# Autodesk Inventor assembly: ElectricalBoxAssembly
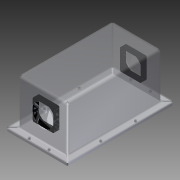
[picture p0: Inventor's stored thumbnail of the model, 180x180]
Saved by Autodesk Inventor 2015 (Build 190159000, 159)
## iProperties
Created: 2015-05-12
Part Number: ElectricalBoxAssembly
Document SubType Name: Assembly
Designer: carpenma
Author: carpenma
## Documents named in this file (4)
- C:\Users\carpe_000\Documents\GitHub\PFPRobot\Mechanical\Drivetrain WIth Cart\Electrical Board-Box\ElectricalBoxAssembly.iam
- C:\Users\carpe_000\Documents\GitHub\PFPRobot\Mechanical\Drivetrain WIth Cart\Electrical Board-Box\60mm Fan Footprint.ipt
- C:\Users\carpe_000\Documents\GitHub\PFPRobot\Mechanical\Drivetrain WIth Cart\Electrical Board-Box\Cover.ipt
- C:\Users\carpe_000\Documents\GitHub\PFPRobot\Mechanical\Drivetrain WIth Cart\Electrical Board-Box\Base.ipt
## Components (4 placed, 3 different names)
1. 60mm Fan Footprint:1 — Mate:1
2. Cover:1 — Mate:1, Mate:2, Mate:3, Mate:4, Mate:5
3. 60mm Fan Footprint:2 — Mate:2
4. Base:1 — Mate:3, Mate:4, Mate:5
## Relationships (5: Mate 5)
- Mate:1: 60mm Fan Footprint:1 ↔ Cover:1
- Mate:2: Cover:1 ↔ 60mm Fan Footprint:2
- Mate:3: Cover:1 ↔ Base:1
- Mate:4: Cover:1 ↔ Base:1
- Mate:5: Cover:1 ↔ Base:1
